# Autodesk Inventor assembly: 5008_Motor
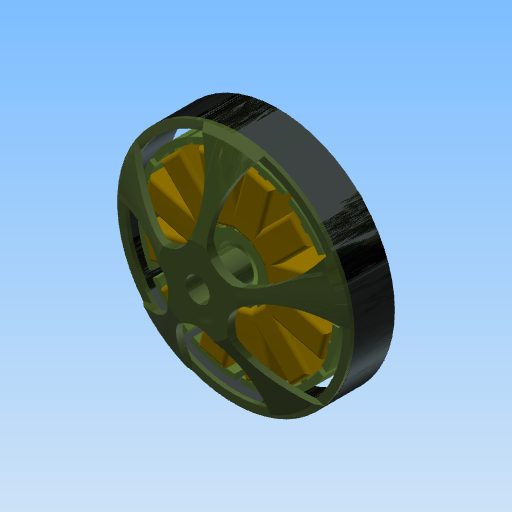
[picture p0: Inventor's stored thumbnail of the model, 512x512]
Saved by Autodesk Inventor 2020.2 (Build 242310000, 310)
## iProperties
Created: 2018-11-06
Part Number: 5008_Motor
Document SubType Name: Assembly
Designer: paulg
Author: paulg
## Documents named in this file (4)
- D:\Projects\MiniBot\CAD\cycloidal gear\source\5008_Motor.iam
- D:\Projects\MiniBot\CAD\cycloidal gear\source\motor 6809 flux.ipt
- D:\Projects\MiniBot\CAD\cycloidal gear\source\motor 6809 stator.ipt
- D:\Projects\MiniBot\CAD\cycloidal gear\source\motor 6809 top.ipt
## Components (3 placed, 3 different names)
1. motor 6809 flux:1 — Insert:1
2. motor 6809 stator:1 — Insert:2
3. motor 6809 top:1 — Insert:1, Insert:2
## Relationships (2: Insert 2)
- Insert:1: motor 6809 flux:1 ↔ motor 6809 top:1
- Insert:2: motor 6809 stator:1 ↔ motor 6809 top:1
